# Autodesk Inventor assembly: Trunk_chest_frame
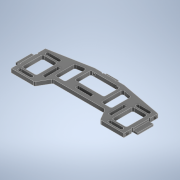
[picture p0: Inventor's stored thumbnail of the model, 180x180]
Saved by Autodesk Inventor 2022.3 (Build 263350000, 350)
## iProperties
Created: 2023-05-08
Part Number: Trunk_chest_frame
Document SubType Name: Assembly
Designer: Masato Kubotera
Author: Masato Kubotera
## Documents named in this file (3)
- C:\Users\Masato\Documents\Inventor\Inventor for CIT Brains\SUSTAINA-OP - mod\UpperBody\Trunk\Trunk_chest_frame.iam
- C:\Users\Masato\Documents\Inventor\Inventor for CIT Brains\SUSTAINA-OP - mod\UpperBody\Trunk\Trunk_chest_frame.ipt
- C:\Users\Masato\Documents\Inventor\Inventor for CIT Brains\SUSTAINA-OP - mod\ReadyMade\InsertNut\IRU-304S.ipt
## Components (7 placed, 2 different names)
1. Trunk_chest_frame:1 — Flush:1, Flush:2, Flush:3, Insert:1, Insert:2, Insert:3, Insert:4, Insert:5, Insert:6
2. IRU-304S:1 — Insert:1
3. IRU-304S:2 — Insert:2
4. IRU-304S:3 — Insert:3
5. IRU-304S:4 — Insert:4
6. IRU-304S:5 — Insert:5
7. IRU-304S:6 — Insert:6
## Relationships (9: Insert 6, Flush 3)
- Flush:1: Trunk_chest_frame:1
- Flush:2: Trunk_chest_frame:1
- Flush:3: Trunk_chest_frame:1
- Insert:1: Trunk_chest_frame:1 ↔ IRU-304S:1
- Insert:2: Trunk_chest_frame:1 ↔ IRU-304S:2
- Insert:3: Trunk_chest_frame:1 ↔ IRU-304S:3
- Insert:4: Trunk_chest_frame:1 ↔ IRU-304S:4
- Insert:5: Trunk_chest_frame:1 ↔ IRU-304S:5
- Insert:6: Trunk_chest_frame:1 ↔ IRU-304S:6
